# Autodesk Inventor assembly: sm_connection
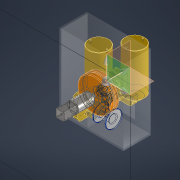
[picture p0: Inventor's stored thumbnail of the model, 180x180]
Saved by Autodesk Inventor 2021 (Build 250183000, 183)
## iProperties
Created: 2021-06-22
Part Number: sm_connection
Document SubType Name: Assembly
Designer: Watchdog
Author: Watchdog
## Documents named in this file (7)
- C:\Users\Watchdog\OneDrive - Flinders\Advn Mech Design Shared\6_Development\2_Design\inventor\securing_mechanism\connection\sm_connection.iam
- C:\Users\Watchdog\OneDrive - Flinders\Advn Mech Design Shared\6_Development\2_Design\inventor\securing_mechanism\connection\gear_khk_SUS1-28J10.ipt
- C:\Users\Watchdog\OneDrive - Flinders\Advn Mech Design Shared\6_Development\2_Design\inventor\securing_mechanism\connection\member_s2c.ipt
- C:\Users\Watchdog\OneDrive - Flinders\Advn Mech Design Shared\6_Development\2_Design\inventor\support\reel\motor.ipt
- C:\Users\Watchdog\OneDrive - Flinders\Advn Mech Design Shared\6_Development\2_Design\inventor\securing_mechanism\connection\box.ipt
- C:\Users\Watchdog\OneDrive - Flinders\Advn Mech Design Shared\6_Development\2_Design\inventor\securing_mechanism\connection\bushing_smConnection.ipt
- C:\Users\Watchdog\OneDrive - Flinders\Advn Mech Design Shared\6_Development\2_Design\inventor\securing_mechanism\connection\secureingReel.ipt
## Components (8 placed, 6 different names)
1. gear_khk_SUS1-28J10:1 — Mate:1, Tangent:1, Flush:2, Flush:3, Mate:5, Mate:8
2. member_s2c:1 — Mate:1, Mate:2, Flush:1, Mate:3, Flush:3, Mate:5, Mate:6
3. motor:1 — Mate:4, Angle:1, Angle:2, Flush:4, Angle:3, Mate:10
4. gear_khk_SUS1-28J10:2 — Tangent:1, Flush:2, Mate:4, Angle:2, Flush:4
5. motor:2 — Angle:3, Mate:11, Mate:12, Mate:13, Mate:14, Angle:4, Mate:15
6. box:1 — Mate:6, Mate:7, Mate:9, Mate:10, Mate:11, Mate:12, Mate:13
7. bushing_smConnection:1 — Mate:7, Mate:8, Mate:9
8. secureingReel:1 — Mate:14, Angle:4, Mate:15
## Relationships (24: Mate 15, Flush 4, Angle 4, Tangent 1)
- Mate:1: gear_khk_SUS1-28J10:1 ↔ member_s2c:1
- Mate:2: member_s2c:1
- Flush:1: member_s2c:1
- Mate:3: member_s2c:1
- Tangent:1: gear_khk_SUS1-28J10:1 ↔ gear_khk_SUS1-28J10:2
- Flush:2: gear_khk_SUS1-28J10:1 ↔ gear_khk_SUS1-28J10:2
- Flush:3: gear_khk_SUS1-28J10:1 ↔ member_s2c:1
- Mate:4: motor:1 ↔ gear_khk_SUS1-28J10:2
- Angle:1 (0 deg): motor:1
- Angle:2 (180 deg): motor:1 ↔ gear_khk_SUS1-28J10:2
- Flush:4: motor:1 ↔ gear_khk_SUS1-28J10:2
- Mate:5: gear_khk_SUS1-28J10:1 ↔ member_s2c:1
- Mate:6: member_s2c:1 ↔ box:1
- Mate:7: box:1 ↔ bushing_smConnection:1
- Mate:8: gear_khk_SUS1-28J10:1 ↔ bushing_smConnection:1
- Mate:9: box:1 ↔ bushing_smConnection:1
- Angle:3 (0 deg): motor:1 ↔ motor:2
- Mate:10: motor:1 ↔ box:1
- Mate:11: motor:2 ↔ box:1
- Mate:12: motor:2 ↔ box:1
- Mate:13: motor:2 ↔ box:1
- Mate:14: motor:2 ↔ secureingReel:1
- Angle:4 (180 deg): motor:2 ↔ secureingReel:1
- Mate:15: motor:2 ↔ secureingReel:1
